# Autodesk Inventor assembly: 前足
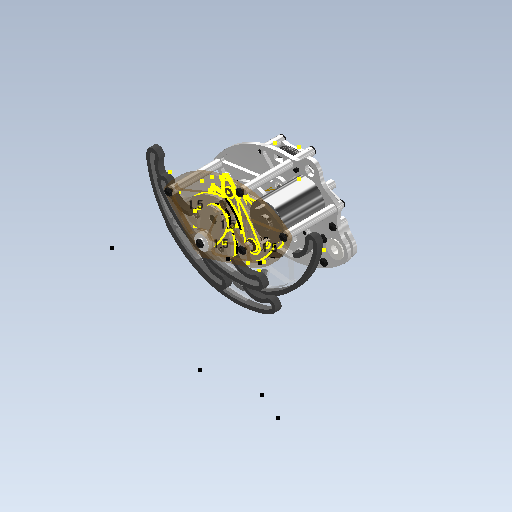
[picture p0: Inventor's stored thumbnail of the model, 512x512]
Saved by Autodesk Inventor 2020.4 (Build 244396000, 396)
## iProperties
Created: 2021-02-23
Part Number: 前足
Document SubType Name: Assembly
Designer: AA19065
Mass: 274.517 g
Surface Area: 1202.78 cm^2
Volume: 103.512 cm^3
Density: 2.65204 g/cm^3
Author: AA19065
## Documents named in this file (24)
- C:\Users\happy\OneDrive\ドキュメント\賢一ファイル\SRDC\試作10-2\アセンブリ\前足.iam
- C:\Users\happy\OneDrive\ドキュメント\賢一ファイル\SRDC\試作10-2\フレーム\前足内側フレームv2.ipt
- C:\Users\happy\OneDrive\ドキュメント\賢一ファイル\SRDC\試作10-2\アセンブリ\脚クランク.iam
- C:\Users\happy\OneDrive\ドキュメント\賢一ファイル\SRDC\試作10-2\軸受け\オイレスw5f12-14n.ipt
- C:\Users\happy\OneDrive\ドキュメント\賢一ファイル\SRDC\試作10-2\スペーサ\40mm.ipt
- C:\Users\happy\OneDrive\ドキュメント\賢一ファイル\SRDC\試作10-2\フレーム\前足外側フレームv2.ipt
- C:\Users\happy\OneDrive\ドキュメント\賢一ファイル\SRDC\試作10-2\軸受け\φ6φ12ベアリングa.ipt
- C:\Users\happy\OneDrive\ドキュメント\賢一ファイル\SRDC\試作10-2\モータ\RS-380.ipt
- C:\Users\happy\OneDrive\ドキュメント\賢一ファイル\SRDC\試作10-2\モータ\モータマウントv2.ipt
- C:\Users\happy\OneDrive\ドキュメント\賢一ファイル\SRDC\試作10-2\軸受け\φ4φ8ベアリングa.ipt
- C:\Users\happy\OneDrive\ドキュメント\賢一ファイル\SRDC\試作10-2\ピン\φ4ピン　L20.ipt
- C:\Users\happy\OneDrive\ドキュメント\賢一ファイル\SRDC\試作10-2\アセンブリ\脚ギア1段目.iam
- C:\Users\happy\OneDrive\ドキュメント\賢一ファイル\SRDC\試作10-2\ギア\ピニオン10.ipt
- C:\Users\happy\OneDrive\ドキュメント\賢一ファイル\SRDC\試作10-2\ギア\m1z60.ipt
- C:\Users\happy\OneDrive\ドキュメント\賢一ファイル\SRDC\試作10-2\ギア\脚ギアマウントv3.ipt
- C:\Users\happy\OneDrive\ドキュメント\賢一ファイル\SRDC\試作10-2\脚クランク\原動節v2\原動節ギア接続部v2.ipt
- C:\Users\happy\OneDrive\ドキュメント\賢一ファイル\SRDC\試作10-2\ねじ\M3ボタンボルト8.ipt
- C:\Users\happy\OneDrive\ドキュメント\賢一ファイル\SRDC\試作10-2\スペーサ\12mm.ipt
- C:\Users\happy\OneDrive\ドキュメント\賢一ファイル\SRDC\試作10-2\ねじ\M3ボタンボルト18.ipt
- C:\Users\happy\OneDrive\ドキュメント\賢一ファイル\SRDC\試作10-2\ねじ\m3皿ネジ12.ipt
- C:\Users\happy\OneDrive\ドキュメント\賢一ファイル\SRDC\試作10-2\フレーム\前足フレーム補助パーツ.ipt
- C:\Users\happy\OneDrive\ドキュメント\賢一ファイル\SRDC\試作10-2\ねじ\m2.6 6mm キャップボルト.ipt
- C:\Users\happy\OneDrive\ドキュメント\賢一ファイル\SRDC\試作10-2\ねじ\M3ボタンボルト20.ipt
- C:\Users\happy\OneDrive\ドキュメント\賢一ファイル\SRDC\試作10-2\スペーサ\18mm.ipt
## Components (45 placed, 23 different names)
1. 前足内側フレームv2:1 — 挿入:2, 挿入:3, 挿入:4, 挿入:5, 挿入:6, 挿入:12, 挿入:13, 挿入:14, 挿入:37, 挿入:38, 挿入:43, 挿入:44, 挿入:47, 挿入:52, 挿入:53, 挿入:54, 挿入:58, 挿入:59, 挿入:60, 挿入:65
2. 脚クランク:1 [sub-assembly] — 挿入:1, メイト:1, 挿入:30, 挿入:31, 挿入:32
3. オイレスw5f12-14n:1 — 挿入:1, 挿入:2
4. 40mm:1 — 挿入:4, 挿入:7
5. 40mm:2 — 挿入:3, メイト:1
6. 40mm:4 — 挿入:6
7. 40mm:5 — 挿入:5, 挿入:8
8. 前足外側フレームv2:1 — 挿入:7, 挿入:8, 挿入:9, 挿入:33, 挿入:34, 挿入:35, 挿入:36
9. φ6φ12ベアリングa:1 — 挿入:9
10. RS-380:1 — 挿入:10, 挿入:11, 挿入:15
11. モータマウントv2:1 — 挿入:10, 挿入:11, 挿入:12, 挿入:13, 挿入:56, 挿入:57, 挿入:61, 挿入:62, 挿入:63
12. φ4φ8ベアリングa:1 — 挿入:14, メイト:3, フラッシュ:1, メイト:4
13. φ4φ8ベアリングa:2 — メイト:5, 挿入:29
14. φ4ピン　L20:1 — メイト:2, メイト:3, フラッシュ:1, メイト:5
15. 脚ギア1段目:1 [sub-assembly] — メイト:2, メイト:4
16. ピニオン10:1 — 挿入:15
17. m1z60:1 — 挿入:32, メイト:6
18. 脚ギアマウントv3:1 — 挿入:29, 挿入:46, 挿入:49, 挿入:50, 挿入:64
19. 原動節ギア接続部v2:1 — 挿入:30, 挿入:31, メイト:6, 挿入:51
20. M3ボタンボルト8:1 — 挿入:33
21. M3ボタンボルト8:2 — 挿入:34
22. M3ボタンボルト8:3 — 挿入:35
23. M3ボタンボルト8:4 — 挿入:36
24. M3ボタンボルト8:5 — 挿入:37
25. M3ボタンボルト8:6 — 挿入:38
26. 12mm:1 — 挿入:47
27. 12mm:2 — 挿入:43, 挿入:46
28. 12mm:3 — 挿入:44
29. M3ボタンボルト18:1 — 挿入:49
30. M3ボタンボルト18:2 — 挿入:50
31. m3皿ネジ12:1 — 挿入:51
32. φ6φ12ベアリングa:2 — 挿入:55
33. 前足フレーム補助パーツ:1 — 挿入:52, 挿入:53, 挿入:55
34. φ6φ12ベアリングa:3 — 挿入:54
35. M3ボタンボルト8:7 — 挿入:56
36. M3ボタンボルト8:8 — 挿入:57
37. M3ボタンボルト8:9
38. M3ボタンボルト8:10 — 挿入:59
39. M3ボタンボルト8:11 — 挿入:58
40. M3ボタンボルト8:12 — 挿入:60
41. M3ボタンボルト8:13 — 挿入:61
42. m2.6 6mm キャップボルト:1 — 挿入:62
43. m2.6 6mm キャップボルト:2 — 挿入:63
44. M3ボタンボルト20:1 — 挿入:64
45. 18mm:1 — 挿入:65
## Relationships (53: Insert 46, Mate 6, Flush 1)
- 挿入:1 [Insert]: 脚クランク:1 ↔ オイレスw5f12-14n:1
- 挿入:2 [Insert] (0.5 mm): 前足内側フレームv2:1 ↔ オイレスw5f12-14n:1
- 挿入:3 [Insert]: 前足内側フレームv2:1 ↔ 40mm:2
- メイト:1 [Mate]: 脚クランク:1 ↔ 40mm:2
- 挿入:4 [Insert]: 前足内側フレームv2:1 ↔ 40mm:1
- 挿入:5 [Insert]: 前足内側フレームv2:1 ↔ 40mm:5
- 挿入:6 [Insert]: 前足内側フレームv2:1 ↔ 40mm:4
- 挿入:7 [Insert]: 40mm:1 ↔ 前足外側フレームv2:1
- 挿入:8 [Insert]: 40mm:5 ↔ 前足外側フレームv2:1
- 挿入:9 [Insert]: 前足外側フレームv2:1 ↔ φ6φ12ベアリングa:1
- 挿入:10 [Insert]: RS-380:1 ↔ モータマウントv2:1
- 挿入:11 [Insert]: RS-380:1 ↔ モータマウントv2:1
- 挿入:12 [Insert]: 前足内側フレームv2:1 ↔ モータマウントv2:1
- 挿入:13 [Insert]: 前足内側フレームv2:1 ↔ モータマウントv2:1
- 挿入:14 [Insert]: 前足内側フレームv2:1 ↔ φ4φ8ベアリングa:1
- メイト:2 [Mate]: φ4ピン　L20:1 ↔ 脚ギア1段目:1
- メイト:3 [Mate]: φ4φ8ベアリングa:1 ↔ φ4ピン　L20:1
- フラッシュ:1 [Flush]: φ4φ8ベアリングa:1 ↔ φ4ピン　L20:1
- 挿入:15 [Insert] (1 mm): RS-380:1 ↔ ピニオン10:1
- メイト:4 [Mate] (2 mm): φ4φ8ベアリングa:1 ↔ 脚ギア1段目:1
- メイト:5 [Mate]: φ4φ8ベアリングa:2 ↔ φ4ピン　L20:1
- 挿入:29 [Insert]: φ4φ8ベアリングa:2 ↔ 脚ギアマウントv3:1
- 挿入:30 [Insert]: 脚クランク:1 ↔ 原動節ギア接続部v2:1
- 挿入:31 [Insert]: 脚クランク:1 ↔ 原動節ギア接続部v2:1
- 挿入:32 [Insert]: 脚クランク:1 ↔ m1z60:1
- メイト:6 [Mate]: m1z60:1 ↔ 原動節ギア接続部v2:1
- 挿入:33 [Insert]: 前足外側フレームv2:1 ↔ M3ボタンボルト8:1
- 挿入:34 [Insert]: 前足外側フレームv2:1 ↔ M3ボタンボルト8:2
- 挿入:35 [Insert]: 前足外側フレームv2:1 ↔ M3ボタンボルト8:3
- 挿入:36 [Insert]: 前足外側フレームv2:1 ↔ M3ボタンボルト8:4
- 挿入:37 [Insert]: 前足内側フレームv2:1 ↔ M3ボタンボルト8:5
- 挿入:38 [Insert]: 前足内側フレームv2:1 ↔ M3ボタンボルト8:6
- 挿入:43 [Insert]: 前足内側フレームv2:1 ↔ 12mm:2
- 挿入:44 [Insert]: 前足内側フレームv2:1 ↔ 12mm:3
- 挿入:46 [Insert]: 脚ギアマウントv3:1 ↔ 12mm:2
- 挿入:47 [Insert]: 前足内側フレームv2:1 ↔ 12mm:1
- 挿入:49 [Insert]: 脚ギアマウントv3:1 ↔ M3ボタンボルト18:1
- 挿入:50 [Insert]: 脚ギアマウントv3:1 ↔ M3ボタンボルト18:2
- 挿入:51 [Insert]: 原動節ギア接続部v2:1 ↔ m3皿ネジ12:1
- 挿入:52 [Insert]: 前足内側フレームv2:1 ↔ 前足フレーム補助パーツ:1
- 挿入:53 [Insert]: 前足内側フレームv2:1 ↔ 前足フレーム補助パーツ:1
- 挿入:54 [Insert]: 前足内側フレームv2:1 ↔ φ6φ12ベアリングa:3
- 挿入:55 [Insert]: φ6φ12ベアリングa:2 ↔ 前足フレーム補助パーツ:1
- 挿入:56 [Insert]: モータマウントv2:1 ↔ M3ボタンボルト8:7
- 挿入:57 [Insert]: モータマウントv2:1 ↔ M3ボタンボルト8:8
- 挿入:58 [Insert]: 前足内側フレームv2:1 ↔ M3ボタンボルト8:11
- 挿入:59 [Insert]: 前足内側フレームv2:1 ↔ M3ボタンボルト8:10
- 挿入:60 [Insert]: 前足内側フレームv2:1 ↔ M3ボタンボルト8:12
- 挿入:61 [Insert]: モータマウントv2:1 ↔ M3ボタンボルト8:13
- 挿入:62 [Insert]: モータマウントv2:1 ↔ m2.6 6mm キャップボルト:1
- 挿入:63 [Insert]: モータマウントv2:1 ↔ m2.6 6mm キャップボルト:2
- 挿入:64 [Insert]: 脚ギアマウントv3:1 ↔ M3ボタンボルト20:1
- 挿入:65 [Insert]: 前足内側フレームv2:1 ↔ 18mm:1
